# Autodesk Inventor assembly: FinalCarro
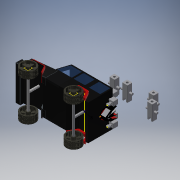
[picture p0: Inventor's stored thumbnail of the model, 180x180]
Saved by Autodesk Inventor 2017 (Build 210142000, 142)
## iProperties
Part Number: FinalCarro
Material: Genérico
Document SubType Name: Assembly
Designer: Ghost
Author: Ghost
## Documents named in this file (8)
- C:\Users\Ghost\Desktop\UVG Semestre 8\Dibujo Mecanico\ProyectoTransformer\FinalCarro.iam
- C:\Users\Ghost\Desktop\UVG Semestre 8\Dibujo Mecanico\ProyectoTransformer\ProyectoTransformer\Bumper.ipt
- C:\Users\Ghost\Desktop\UVG Semestre 8\Dibujo Mecanico\ProyectoTransformer\ProyectoTransformer\CabezaCarro.ipt
- C:\Users\Ghost\Desktop\UVG Semestre 8\Dibujo Mecanico\ProyectoTransformer\ProyectoTransformer\PuertaMarco.iam
- C:\Users\Ghost\Desktop\UVG Semestre 8\Dibujo Mecanico\ProyectoTransformer\ProyectoTransformer\llanta.ipt
- C:\Users\Ghost\Desktop\UVG Semestre 8\Dibujo Mecanico\ProyectoTransformer\ProyectoTransformer\Hombro.ipt
- C:\Users\Ghost\Desktop\UVG Semestre 8\Dibujo Mecanico\ProyectoTransformer\ProyectoTransformer\Union pie.ipt
- C:\Users\Ghost\Desktop\UVG Semestre 8\Dibujo Mecanico\ProyectoTransformer\ProyectoTransformer\Ante pierna.ipt
## Components (19 placed, 7 different names)
1. Bumper:1 — Insertar:1, Insertar:2, Insertar:5, Insertar:6
2. CabezaCarro:1 — Coincidencia:1, Insertar:3
3. PuertaMarco:1 [sub-assembly] — Insertar:1, Insertar:2, Coincidencia:1, Insertar:3, Insertar:4, Insertar:7, Insertar:8, Insertar:9, Insertar:10, Insertar:11
4. llanta:1 — Insertar:5
5. llanta:2 — Insertar:6
6. llanta:3 — Insertar:7
7. llanta:4 — Insertar:4
8. Hombro:1 — Insertar:8, Insertar:14
9. Hombro:2 — Insertar:9, Insertar:12
10. Hombro:3 — Insertar:11, Insertar:15
11. Hombro:4 — Insertar:10, Insertar:13
12. Union pie:1 — Insertar:15
13. Union pie:2 — Insertar:14
14. Union pie:3 — Insertar:13
15. Union pie:4 — Insertar:12
16. Ante pierna:1
17. Ante pierna:2
18. Ante pierna:3
19. Ante pierna:4
## Relationships (16: Insert 15, Mate 1)
- Insertar:1: Bumper:1 ↔ PuertaMarco:1
- Insertar:2: Bumper:1 ↔ PuertaMarco:1
- Coincidencia:1 [Mate]: CabezaCarro:1 ↔ PuertaMarco:1
- Insertar:3: CabezaCarro:1 ↔ PuertaMarco:1
- Insertar:4: PuertaMarco:1 ↔ llanta:4
- Insertar:5: Bumper:1 ↔ llanta:1
- Insertar:6: Bumper:1 ↔ llanta:2
- Insertar:7: PuertaMarco:1 ↔ llanta:3
- Insertar:8: PuertaMarco:1 ↔ Hombro:1
- Insertar:9: PuertaMarco:1 ↔ Hombro:2
- Insertar:10: PuertaMarco:1 ↔ Hombro:4
- Insertar:11: PuertaMarco:1 ↔ Hombro:3
- Insertar:12: Hombro:2 ↔ Union pie:4
- Insertar:13: Hombro:4 ↔ Union pie:3
- Insertar:14: Hombro:1 ↔ Union pie:2
- Insertar:15: Hombro:3 ↔ Union pie:1
